# Autodesk Inventor assembly: Assembly_Motorcoupling_Nema_M3_Selfcentering
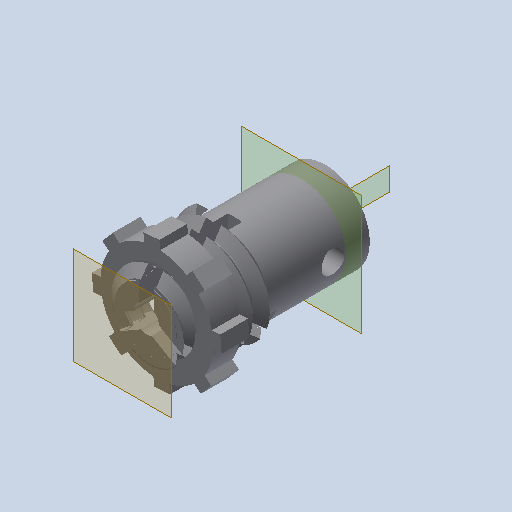
[picture p0: Inventor's stored thumbnail of the model, 512x512]
Saved by Autodesk Inventor 2022 (Build 260153000, 153)
## iProperties
Created: 2021-09-11
Part Number: Assembly_Motorcoupling_Nema_M3_Selfcentering
Document SubType Name: Assembly
Designer: diederichbenedict
Author: diederichbenedict
## Documents named in this file (3)
- C:\Users\diederichbenedict\Dropbox\Dokumente\Promotion\PROJECTS\UC2\02_CAD\INVENTOR\uc2_v3\Assembly_Motorcoupling_Nema_M3_Selfcentering.iam
- C:\Users\diederichbenedict\Dropbox\Dokumente\Promotion\PROJECTS\UC2\02_CAD\INVENTOR\uc2_v3\00_coupler_5_3_nema_screw.ipt
- C:\Users\diederichbenedict\Dropbox\Dokumente\Promotion\PROJECTS\UC2\02_CAD\INVENTOR\uc2_v3\00_coupler_5_3_nema_screw_nut.ipt
## Components (2 placed, 2 different names)
1. 00_coupler_5_3_nema_screw:1 — Mate:1
2. 00_coupler_5_3_nema_screw_nut:1 — Mate:1
## Relationships (1: Mate 1)
- Mate:1: 00_coupler_5_3_nema_screw:1 ↔ 00_coupler_5_3_nema_screw_nut:1
